# Autodesk Inventor assembly: Top Bar
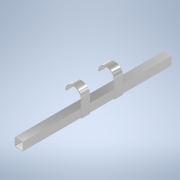
[picture p0: Inventor's stored thumbnail of the model, 180x180]
Saved by Autodesk Inventor 2020 (Build 240168000, 168)
## iProperties
Created: 2020-01-30
Part Number: Top Bar
Document SubType Name: Assembly
Designer: autum
Author: autum
## Documents named in this file (3)
- C:\Users\autum\Google Drive\Iron Riders 4180 (Roosevelt Robotics)\2019-2020\Build_Design\Robot 2020 (1)\Climber\Top Bar.iam
- C:\Users\autum\Google Drive\Iron Riders 4180 (Roosevelt Robotics)\2019-2020\Build_Design\Robot 2020 (1)\Climber\Top Bar.ipt
- C:\Users\autum\Google Drive\Iron Riders 4180 (Roosevelt Robotics)\2019-2020\Build_Design\Robot 2020 (1)\Climber\Hook 2.0.ipt
## Components (3 placed, 2 different names)
1. Top Bar:1 — Mate:1, Mate:2, Flush:1, Flush:2, Flush:3
2. Hook 2.0:1 — Mate:1, Flush:2, Mate:3
3. Hook 2.0:2 — Mate:2, Flush:1, Mate:3, Flush:3
## Relationships (6: Mate 3, Flush 3)
- Mate:1: Top Bar:1 ↔ Hook 2.0:1
- Mate:2: Top Bar:1 ↔ Hook 2.0:2
- Flush:1: Top Bar:1 ↔ Hook 2.0:2
- Flush:2: Top Bar:1 ↔ Hook 2.0:1
- Mate:3 (76.2 mm): Hook 2.0:1 ↔ Hook 2.0:2
- Flush:3 (177.8 mm): Top Bar:1 ↔ Hook 2.0:2
